# Autodesk Inventor assembly: MG-Dribbler Seite
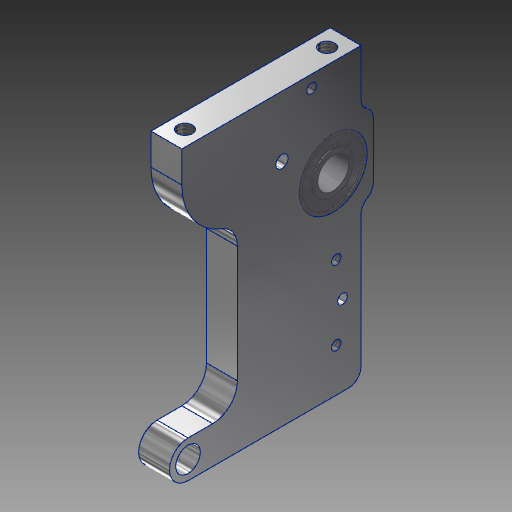
[picture p0: Inventor's stored thumbnail of the model, 512x512]
Saved by Autodesk Inventor 2019.4 (Build 234330000, 330)
## iProperties
Part Number: MG-Dribbler Seite
Material: Generisch
Document SubType Name: Assembly
Designer: rYan
Mass: 16.4982 g
Surface Area: 37.7813 cm^2
Volume: 5.42517 cm^3
Density: 3.04104 g/cm^3
Author: rYan
## Documents named in this file (3)
- D:\TIGERsGIT\Hardware\mechanik\2020\Inventor\Robot\Dribbler\MG-Dribbler Seite.iam
- D:\TIGERsGIT\Hardware\mechanik\2020\Inventor\Robot\Dribbler\Dribbler Seite.ipt
- D:\TIGERsGIT\Hardware\mechanik\2020\Inventor\Purchased Parts\Kugellager 685-ZZ-C3.ipt
## Components (2 placed, 2 different names)
1. Dribbler Seite:1 — Einfügen:1
2. Kugellager 685-ZZ-C3:1 — Einfügen:1
## Relationships (1: Insert 1)
- Einfügen:1 [Insert]: Dribbler Seite:1 ↔ Kugellager 685-ZZ-C3:1
